# Autodesk Inventor assembly: independent_wheel_pair
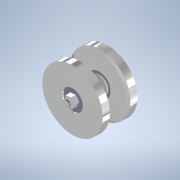
[picture p0: Inventor's stored thumbnail of the model, 180x180]
Saved by Autodesk Inventor 2020.3 (Build 243373000, 373)
## iProperties
Created: 2021-03-25
Part Number: independent_wheel_pair
Document SubType Name: Assembly
Designer: patry
Mass: 73.5609 g
Surface Area: 155.822 cm^2
Volume: 27.2448 cm^3
Density: 2.7 g/cm^3
Author: patry
## Documents named in this file (6)
- C:\Users\patry\Desktop\Semestr 7\Inzynierka\Projekt inventor\Ariadna_inzynierka\Workspaces\Obszar roboczy\Obszar roboczy\Naped\Zawieszenie_v3\independent_wheel_pair.iam
- C:\Users\patry\Desktop\Semestr 7\Inzynierka\Projekt inventor\Ariadna_inzynierka\Workspaces\Obszar roboczy\Obszar roboczy\Naped\Kola\single_wheel.iam
- C:\Users\patry\Desktop\Semestr 7\Inzynierka\Projekt inventor\Ariadna_inzynierka\Workspaces\Obszar roboczy\Obszar roboczy\Naped\Sruby\M5_nut_5mm.ipt
- C:\Users\patry\Desktop\Semestr 7\Inzynierka\Projekt inventor\Ariadna_inzynierka\Workspaces\Obszar roboczy\Obszar roboczy\Naped\Sruby\M5_pad.ipt
- C:\Users\patry\Desktop\Semestr 7\Inzynierka\Projekt inventor\Ariadna_inzynierka\Workspaces\Obszar roboczy\Obszar roboczy\Naped\Sruby\M5_40_shaft.ipt
- M5_shaft.ipt
## Components (7 placed, 4 different names)
1. single_wheel:1 [sub-assembly] — Zestawiające:1, Zestawiające:2, Zestawiające:6, Zestawiające:10, Zestawiające:13, Zestawiające:14, Równoległe:1
2. single_wheel:2 [sub-assembly] — Zestawiające:1, Zestawiające:2, Zestawiające:7, Zestawiające:15, Zestawiające:17
3. M5_nut_5mm:1 — Zestawiające:6, Zestawiające:13, Zestawiające:16, Zestawiające:18
4. M5_pad:1 — Zestawiające:7, Zestawiające:15
5. M5_nut_5mm:4 — Zestawiające:16, Zestawiające:17
6. M5_pad:2 — Zestawiające:10, Zestawiające:14
7. M5_shaft:1 — Zestawiające:18, Równoległe:1
## Relationships (12: Mate 11, Flush 1)
- Zestawiające:1 [Mate] (15 mm): single_wheel:1 ↔ single_wheel:2
- Zestawiające:2 [Mate]: single_wheel:1 ↔ single_wheel:2
- Zestawiające:6 [Mate]: single_wheel:1 ↔ M5_nut_5mm:1
- Zestawiające:7 [Mate] (-0.25 mm): single_wheel:2 ↔ M5_pad:1
- Zestawiające:10 [Mate] (-0.25 mm): single_wheel:1 ↔ M5_pad:2
- Zestawiające:13 [Mate]: single_wheel:1 ↔ M5_nut_5mm:1
- Zestawiające:14 [Mate]: single_wheel:1 ↔ M5_pad:2
- Zestawiające:15 [Mate]: single_wheel:2 ↔ M5_pad:1
- Zestawiające:16 [Mate]: M5_nut_5mm:1 ↔ M5_nut_5mm:4
- Zestawiające:17 [Mate]: single_wheel:2 ↔ M5_nut_5mm:4
- Zestawiające:18 [Mate]: M5_nut_5mm:1 ↔ M5_shaft:1
- Równoległe:1 [Flush] (5.5 mm): single_wheel:1 ↔ M5_shaft:1
